# Autodesk Inventor assembly: Assembly1
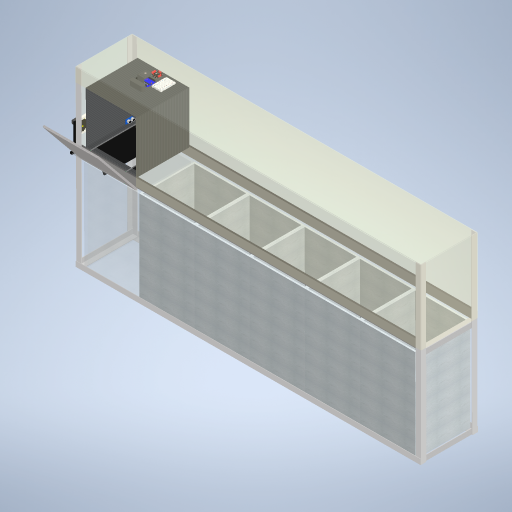
[picture p0: Inventor's stored thumbnail of the model, 512x512]
Saved by Autodesk Inventor 2024 (Build 280153000, 153)
## iProperties
Created: 2024-04-05
Part Number: Assembly1
Document SubType Name: Assembly
Designer: ASUS
Author: ASUS
## Documents named in this file (27)
- D:\Temp\Kuliah\Skripsi\CAD\CAD 2\Assembly1.iam
- D:\Temp\Kuliah\Skripsi\CAD\CAD 2\frame.ipt
- D:\Temp\Kuliah\Skripsi\CAD\CAD 2\frame side.ipt
- D:\Temp\Kuliah\Skripsi\CAD\CAD 2\temporary.ipt
- D:\Temp\Kuliah\Skripsi\CAD\Source\Rack and Pinion\pinion gear 3mm middle.ipt
- D:\Temp\Kuliah\Skripsi\CAD\Source\Rack and Pinion\rack gear.ipt
- D:\Temp\Kuliah\Skripsi\CAD\Source\Rack and Pinion\rack gear 2.ipt
- D:\Temp\Kuliah\Skripsi\CAD\CAD 2\track.ipt
- D:\Temp\Kuliah\Skripsi\CAD\CAD 2\bracket-temporary-1.ipt
- D:\Temp\Kuliah\Skripsi\CAD\CAD 2\bracket-temporary-2.ipt
- D:\Temp\Kuliah\Skripsi\CAD\CAD 2\container.ipt
- D:\Temp\Kuliah\Skripsi\CAD\CAD 2\opener.ipt
- D:\Temp\Kuliah\Skripsi\CAD\CAD 2\opener_main.ipt
- D:\Temp\Kuliah\Skripsi\CAD\Source\Rack and Pinion\rack_gear_main.ipt
- D:\Temp\Kuliah\Skripsi\CAD\CAD 2\cover side.ipt
- D:\Temp\Kuliah\Skripsi\CAD\CAD 2\cover back.ipt
- D:\Temp\Kuliah\Skripsi\CAD\CAD 2\cover front.ipt
- D:\Temp\Kuliah\Skripsi\CAD\CAD 2\cover top.ipt
- D:\Temp\Kuliah\Skripsi\CAD\CAD 2\servo_mount.ipt
- D:\Temp\Kuliah\Skripsi\CAD\Source\Servo MG996R\MG996R Servo\MG996R Servo.ipt
- D:\Temp\Kuliah\Skripsi\CAD\Source\Arduino Uno\arduino uno.iam
- D:\Temp\Kuliah\Skripsi\CAD\Source\Breadboard\Breadboard 400.ipt
- D:\Temp\Kuliah\Skripsi\CAD\Source\Stepper Driver\Closed Loop Driver Nema 17.ipt
- D:\Temp\Kuliah\Skripsi\CAD\Source\NEMA 17\Assembly1.iam
- D:\Temp\Kuliah\Skripsi\CAD\Source\WebCam\Hikvision_DS-U02.iam
- D:\Temp\Kuliah\Skripsi\CAD\Source\HC-SR04\Grove_Ultrasonic_Sensor_V2.0.iam
- D:\Temp\Kuliah\Skripsi\CAD\CAD 2\stick.ipt
## Components (49 placed, 26 different names)
1. frame:1 — Mate:4, Mate:5, Flush:4, Mate:34, Flush:18, Mate:73, Flush:29, Flush:30, Mate:78, Flush:36, Flush:37, Mate:79
2. frame:2 — Mate:14, Mate:15, Flush:6, Mate:74, Flush:34, Flush:35
3. frame:3 — Mate:2, Mate:3, Flush:3, Mate:6, Mate:8, Mate:46, Mate:52, Flush:31, Flush:32, Mate:80, Flush:38, Flush:39, Mate:82
4. frame:4 — Mate:20, Mate:21, Mate:36, Mate:37, Flush:16, Mate:49, Mate:50, Mate:77
5. frame:5 — Mate:1, Flush:1, Flush:2, Mate:4, Mate:5, Flush:4, Mate:35, Mate:39
6. frame:6 — Mate:1, Flush:1, Flush:2, Mate:2, Mate:3, Flush:3, Mate:7, Flush:14, Flush:15
7. frame:7 — Flush:15, Flush:17, Mate:38
8. frame:8 — Flush:14, Mate:37, Flush:16, Flush:17, Mate:38, Mate:40
9. frame side:1 — Mate:6, Mate:7, Mate:8, Mate:14, Mate:15, Flush:6
10. frame side:2 — Mate:34, Mate:35, Mate:36
11. frame side:3 — Mate:46, Mate:52, Mate:53
12. frame side:4 — Mate:49, Mate:50, Mate:51, Mate:54, Mate:81
13. temporary:1 — Mate:29, Flush:10, Flush:11, Mate:64, Mate:65, Mate:66, Mate:67, Mate:68, Mate:69, Mate:71, Mate:72, Rotational:4, Mate:84, Mate:85, Mate:86, Mate:87, Mate:91, Mate:92, Mate:93, Mate:94, Mate:95, Mate:96
14. container:1 — Mate:43, Mate:44, Flush:21, Flush:22, Flush:26, Flush:27
15. container:2 — Mate:42, Mate:43, Flush:20, Flush:21, Flush:25, Flush:26
16. container:3 — Mate:41, Mate:42, Flush:19, Flush:20, Flush:24, Flush:25
17. container:4 — Mate:39, Mate:40, Flush:18, Mate:41, Flush:19, Flush:24, Mate:51
18. container:5 — Mate:44, Mate:45, Flush:22, Flush:23, Flush:27, Flush:28
19. container:6 — Mate:45, Flush:23, Flush:28, Mate:53
20. track:1 — Mate:20, Mate:21, Mate:24, Flush:9, Mate:28, Mate:54
21. track:2 — Mate:79, Mate:80, Mate:81, Rotational:3
22. bracket-temporary-1:1 — Mate:24, Flush:9, Mate:25, Mate:26, Mate:27
23. bracket-temporary-2:1 — Mate:25, Mate:26, Mate:27, Mate:28, Mate:29, Flush:10, Flush:11, Mate:88
24. pinion gear 3mm middle:1 — Rotational:4
25. rack gear:1 — Mate:69, Mate:72, Mate:98
26. rack gear 2:1 — Mate:68, Mate:71, Mate:99
27. opener:1 — Mate:64, Mate:65
28. opener:2 — Mate:66, Mate:67
29. rack_gear_main:1 — Mate:75, Flush:33, Mate:97
30. pinion gear 3mm middle:2 — Mate:76
31. opener_main:1 — Rotational:3
32. servo_mount:1 — Mate:83, Rigid:1
33. cover side:1 — Mate:74, Flush:31, Flush:32, Mate:75, Flush:33, Mate:76, Mate:83
34. cover side:2 — Mate:73, Flush:29, Flush:30
35. cover back:1 — Mate:77, Flush:34, Flush:35
36. cover front:1 — Mate:78, Flush:36, Flush:37
37. cover top:1 — Flush:38, Flush:39, Mate:82
38. MG996R Servo:1 — Mate:84
39. MG996R Servo:2 — Rigid:1
40. arduino uno:1 [sub-assembly] — Mate:85
41. Breadboard 400:1 — Mate:86
42. Closed Loop Driver Nema 17:1 — Mate:87
43. Assembly1:1 [sub-assembly] — Mate:88
44. Hikvision_DS-U02:1 [sub-assembly] — Mate:95, Mate:96
45. Ultrasonic Ranger V2_0:1 [sub-assembly] — Mate:91, Mate:92
46. Ultrasonic Ranger V2_0:2 [sub-assembly] — Mate:93, Mate:94
47. stick:1 — Mate:97
48. stick:2 — Mate:98
49. stick:3 — Mate:99
## Relationships (107: Mate 70, Flush 34, RevoluteJoint 2, WeldJoint 1)
- Mate:1: frame:5 ↔ frame:6
- Flush:1: frame:5 ↔ frame:6
- Flush:2: frame:5 ↔ frame:6
- Mate:2: frame:3 ↔ frame:6
- Mate:3: frame:3 ↔ frame:6
- Flush:3: frame:3 ↔ frame:6
- Mate:4: frame:1 ↔ frame:5
- Mate:5: frame:1 ↔ frame:5
- Flush:4: frame:1 ↔ frame:5
- Mate:6: frame:3 ↔ frame side:1
- Mate:7: frame:6 ↔ frame side:1
- Mate:8: frame:3 ↔ frame side:1
- Mate:14: frame:2 ↔ frame side:1
- Mate:15: frame:2 ↔ frame side:1
- Flush:6: frame:2 ↔ frame side:1
- Mate:20: frame:4 ↔ track:1
- Mate:21: frame:4 ↔ track:1
- Mate:24: track:1 ↔ bracket-temporary-1:1
- Flush:9 (-10 mm): track:1 ↔ bracket-temporary-1:1
- Mate:25 (10 mm): bracket-temporary-1:1 ↔ bracket-temporary-2:1
- Mate:26 (10 mm): bracket-temporary-1:1 ↔ bracket-temporary-2:1
- Mate:27 (10 mm): bracket-temporary-1:1 ↔ bracket-temporary-2:1
- Mate:28: track:1 ↔ bracket-temporary-2:1
- Mate:29 (13 mm): temporary:1 ↔ bracket-temporary-2:1
- Flush:10 (50 mm): temporary:1 ↔ bracket-temporary-2:1
- Flush:11 (60 mm): temporary:1 ↔ bracket-temporary-2:1
- Mate:34: frame:1 ↔ frame side:2
- Mate:35: frame:5 ↔ frame side:2
- Mate:36: frame:4 ↔ frame side:2
- Flush:14: frame:6 ↔ frame:8
- Flush:15: frame:6 ↔ frame:7
- Mate:37: frame:4 ↔ frame:8
- Flush:16: frame:4 ↔ frame:8
- Flush:17: frame:7 ↔ frame:8
- Mate:38: frame:7 ↔ frame:8
- Mate:39: frame:5 ↔ container:4
- Mate:40: frame:8 ↔ container:4
- Flush:18 (-40 mm): frame:1 ↔ container:4
- Mate:41: container:3 ↔ container:4
- Mate:42: container:2 ↔ container:3
- Mate:43: container:1 ↔ container:2
- Mate:44: container:1 ↔ container:5
- Mate:45: container:5 ↔ container:6
- Flush:19: container:3 ↔ container:4
- Flush:20: container:2 ↔ container:3
- Flush:21: container:1 ↔ container:2
- Flush:22: container:1 ↔ container:5
- Flush:23: container:5 ↔ container:6
- Flush:24: container:3 ↔ container:4
- Flush:25: container:2 ↔ container:3
- Flush:26: container:1 ↔ container:2
- Flush:27: container:1 ↔ container:5
- Flush:28: container:5 ↔ container:6
- Mate:46: frame:3 ↔ frame side:3
- Mate:49: frame:4 ↔ frame side:4
- Mate:50: frame:4 ↔ frame side:4
- Mate:51 (20 mm): frame side:4 ↔ container:4
- Mate:52: frame:3 ↔ frame side:3
- Mate:53 (20 mm): frame side:3 ↔ container:6
- Mate:54: frame side:4 ↔ track:1
- Rotational:3 [RevoluteJoint] (30 mm): track:2 ↔ opener_main:1
- Mate:64: temporary:1 ↔ opener:1
- Mate:65: temporary:1 ↔ opener:1
- Mate:66: temporary:1 ↔ opener:2
- Mate:67: temporary:1 ↔ opener:2
- Mate:68: temporary:1 ↔ rack gear 2:1
- Mate:69: temporary:1 ↔ rack gear:1
- Mate:71 (31 mm): temporary:1 ↔ rack gear 2:1
- Mate:72 (32 mm): temporary:1 ↔ rack gear:1
- Rotational:4 [RevoluteJoint]: temporary:1 ↔ pinion gear 3mm middle:1
- Mate:73: frame:1 ↔ cover side:2
- Flush:29: frame:1 ↔ cover side:2
- Flush:30: frame:1 ↔ cover side:2
- Mate:74: frame:2 ↔ cover side:1
- Flush:31: frame:3 ↔ cover side:1
- Flush:32: frame:3 ↔ cover side:1
- Mate:75: rack_gear_main:1 ↔ cover side:1
- Flush:33: rack_gear_main:1 ↔ cover side:1
- Mate:76: pinion gear 3mm middle:2 ↔ cover side:1
- Mate:77: frame:4 ↔ cover back:1
- Flush:34: frame:2 ↔ cover back:1
- Flush:35: frame:2 ↔ cover back:1
- Mate:78: frame:1 ↔ cover front:1
- Flush:36: frame:1 ↔ cover front:1
- Flush:37: frame:1 ↔ cover front:1
- Mate:79: frame:1 ↔ track:2
- Mate:80: frame:3 ↔ track:2
- Mate:81: frame side:4 ↔ track:2
- Flush:38: frame:3 ↔ cover top:1
- Flush:39: frame:3 ↔ cover top:1
- Mate:82: frame:3 ↔ cover top:1
- Mate:83: servo_mount:1 ↔ cover side:1
- Mate:84: temporary:1 ↔ MG996R Servo:1
- Rigid:1 [WeldJoint]: servo_mount:1 ↔ MG996R Servo:2
- Mate:85: temporary:1 ↔ arduino uno:1
- Mate:86: temporary:1 ↔ Breadboard 400:1
- Mate:87: temporary:1 ↔ Closed Loop Driver Nema 17:1
- Mate:88: bracket-temporary-2:1 ↔ Assembly1:1
- Mate:91: temporary:1 ↔ Ultrasonic Ranger V2_0:1
- Mate:92: temporary:1 ↔ Ultrasonic Ranger V2_0:1
- Mate:93: temporary:1 ↔ Ultrasonic Ranger V2_0:2
- Mate:94: temporary:1 ↔ Ultrasonic Ranger V2_0:2
- Mate:95: temporary:1 ↔ Hikvision_DS-U02:1
- Mate:96: temporary:1 ↔ Hikvision_DS-U02:1
- Mate:97: rack_gear_main:1 ↔ stick:1
- Mate:98: rack gear:1 ↔ stick:2
- Mate:99: rack gear 2:1 ↔ stick:3
